# Autodesk Inventor assembly: Selection_Exit Pipe Assy 3 Lanes
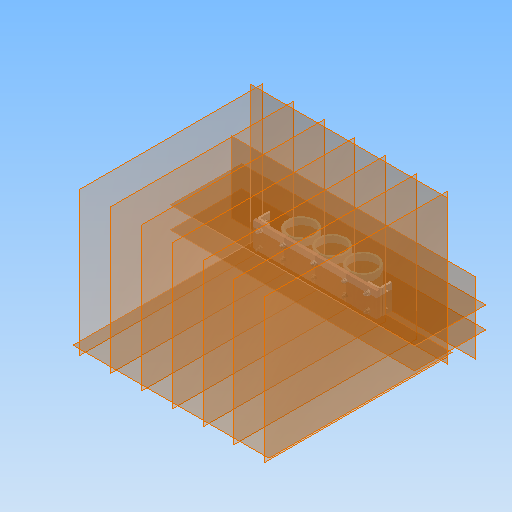
[picture p0: Inventor's stored thumbnail of the model, 512x512]
Saved by Autodesk Inventor 2018.1 (Build 221171000, 171)
## iProperties
Created: 2019-02-11
Part Number: Selection_Exit Pipe Assy 3 Lanes
Document SubType Name: Assembly
Designer: James
Author: James
## Documents named in this file (7)
- C:\Users\admin\Desktop\Ball-Machine\Selection Sort\Selection - 3 Lanes\Selection_Exit Pipe Assy 3 Lanes.iam
- C:\Users\admin\Desktop\Ball-Machine\Prototype CAD\Selection Sort - 40mm\Nyloc Nut - M4.ipt
- C:\Users\admin\Desktop\Ball-Machine\Prototype CAD\Selection Sort - 40mm\Socket Csk Screw - (A2) - M4 x  16.ipt
- C:\Users\admin\Desktop\Ball-Machine\Timing Gate\Timing_Angle Bracket.ipt
- C:\Users\admin\Desktop\Ball-Machine\Prototype CAD\Selection Sort - 40mm\Socket Cap Screw - Standard - (A2) - M4 x 16.ipt
- C:\Users\admin\Desktop\Ball-Machine\Selection Sort\Selection_Exit Pipe.ipt
- C:\Users\admin\Desktop\Ball-Machine\Timing Gate\Timing - 3 Lanes\Timing_Backboard 3 Lanes.ipt
## Components (26 placed, 6 different names)
1. Timing_Backboard 3 Lanes:1 — Flush:18, Tangent:1, Flush:19, Flush:20, Mate:55, Mate:56, Mate:59, Mate:60, Mate:67, Mate:68, Mate:69, Flush:27, Flush:28, Mate:74, Mate:75, Flush:29, Mate:82, Flush:30, Mate:83, Mate:84, Mate:85, Mate:88, Mate:89
2. Timing_Angle Bracket:1 — Mate:67, Mate:68, Mate:69, Flush:27, Flush:28, Mate:70, Mate:71, Mate:72, Mate:73
3. Nyloc Nut - M4:13 — Mate:74, Mate:76
4. Socket Cap Screw - Standard - (A2) - M4 x 16:3 — Mate:72, Mate:73, Mate:77
5. Nyloc Nut - M4:14 — Mate:75, Mate:77
6. Socket Cap Screw - Standard - (A2) - M4 x 16:4 — Mate:70, Mate:71, Mate:76
7. Timing_Angle Bracket:2 — Flush:29, Mate:82, Flush:30, Mate:83
8. Socket Cap Screw - Standard - (A2) - M4 x 16:5 — Mate:87
9. Socket Cap Screw - Standard - (A2) - M4 x 16:6 — Mate:86
10. Nyloc Nut - M4:15 — Mate:84, Mate:87
11. Nyloc Nut - M4:16 — Mate:85, Mate:86
12. Selection_Exit Pipe:1 — Tangent:1, Angle:1, Mate:88, Mate:89, Mate:90
13. Socket Csk Screw - (A2) - M4 x  16:1 — Mate:55, Flush:21, Mate:57, Mate:90
14. Nyloc Nut - M4:2 — Mate:57, Mate:60
15. Nyloc Nut - M4:1 — Mate:58, Mate:59
16. Socket Csk Screw - (A2) - M4 x  16:2 — Flush:21, Mate:56, Mate:58
17. Selection_Exit Pipe:2
18. Socket Csk Screw - (A2) - M4 x  16:3
19. Nyloc Nut - M4:17
20. Nyloc Nut - M4:18
21. Socket Csk Screw - (A2) - M4 x  16:4
22. Selection_Exit Pipe:3
23. Socket Csk Screw - (A2) - M4 x  16:5
24. Nyloc Nut - M4:19
25. Nyloc Nut - M4:20
26. Socket Csk Screw - (A2) - M4 x  16:6
## Component patterns: (3 elements, first: Selection_Exit Pipe:1 + Socket Csk Screw - (A2) - M4 x  16:1 + Nyloc Nut - M4:2 + Nyloc Nut - M4:1 + Socket Csk Screw - (A2) - M4 x  16:2)
## Relationships (43: Mate 30, Flush 11, Tangent 1, Angle 1)
- Flush:11 (-57.5 mm)
- Flush:12 (-5 mm)
- Flush:13 (30 mm)
- Flush:18: Timing_Backboard 3 Lanes:1
- Tangent:1: Timing_Backboard 3 Lanes:1 ↔ Selection_Exit Pipe:1
- Flush:19: Timing_Backboard 3 Lanes:1
- Flush:20: Timing_Backboard 3 Lanes:1
- Mate:55 (-10.3 mm): Timing_Backboard 3 Lanes:1 ↔ Socket Csk Screw - (A2) - M4 x  16:1
- Flush:21: Socket Csk Screw - (A2) - M4 x  16:1 ↔ Socket Csk Screw - (A2) - M4 x  16:2
- Mate:56: Timing_Backboard 3 Lanes:1 ↔ Socket Csk Screw - (A2) - M4 x  16:2
- Mate:57: Socket Csk Screw - (A2) - M4 x  16:1 ↔ Nyloc Nut - M4:2
- Mate:58: Nyloc Nut - M4:1 ↔ Socket Csk Screw - (A2) - M4 x  16:2
- Mate:59: Timing_Backboard 3 Lanes:1 ↔ Nyloc Nut - M4:1
- Mate:60: Timing_Backboard 3 Lanes:1 ↔ Nyloc Nut - M4:2
- Mate:67: Timing_Backboard 3 Lanes:1 ↔ Timing_Angle Bracket:1
- Mate:68: Timing_Backboard 3 Lanes:1 ↔ Timing_Angle Bracket:1
- Mate:69: Timing_Backboard 3 Lanes:1 ↔ Timing_Angle Bracket:1
- Flush:27: Timing_Backboard 3 Lanes:1 ↔ Timing_Angle Bracket:1
- Flush:28: Timing_Backboard 3 Lanes:1 ↔ Timing_Angle Bracket:1
- Mate:70: Timing_Angle Bracket:1 ↔ Socket Cap Screw - Standard - (A2) - M4 x 16:4
- Mate:71: Timing_Angle Bracket:1 ↔ Socket Cap Screw - Standard - (A2) - M4 x 16:4
- Mate:72: Timing_Angle Bracket:1 ↔ Socket Cap Screw - Standard - (A2) - M4 x 16:3
- Mate:73: Timing_Angle Bracket:1 ↔ Socket Cap Screw - Standard - (A2) - M4 x 16:3
- Mate:74: Timing_Backboard 3 Lanes:1 ↔ Nyloc Nut - M4:13
- Mate:75: Timing_Backboard 3 Lanes:1 ↔ Nyloc Nut - M4:14
- Mate:76: Nyloc Nut - M4:13 ↔ Socket Cap Screw - Standard - (A2) - M4 x 16:4
- Mate:77: Socket Cap Screw - Standard - (A2) - M4 x 16:3 ↔ Nyloc Nut - M4:14
- [Mate]: Timing_Angle Bracket:2 ↔ Socket Cap Screw - Standard - (A2) - M4 x 16:6
- [Mate]: Timing_Angle Bracket:2 ↔ Socket Cap Screw - Standard - (A2) - M4 x 16:6
- [Mate]: Timing_Angle Bracket:2 ↔ Socket Cap Screw - Standard - (A2) - M4 x 16:5
- [Mate]: Timing_Angle Bracket:2 ↔ Socket Cap Screw - Standard - (A2) - M4 x 16:5
- Flush:29: Timing_Backboard 3 Lanes:1 ↔ Timing_Angle Bracket:2
- Mate:82: Timing_Backboard 3 Lanes:1 ↔ Timing_Angle Bracket:2
- Flush:30: Timing_Backboard 3 Lanes:1 ↔ Timing_Angle Bracket:2
- Mate:83: Timing_Backboard 3 Lanes:1 ↔ Timing_Angle Bracket:2
- Mate:84: Timing_Backboard 3 Lanes:1 ↔ Nyloc Nut - M4:15
- Mate:85: Timing_Backboard 3 Lanes:1 ↔ Nyloc Nut - M4:16
- Mate:86: Socket Cap Screw - Standard - (A2) - M4 x 16:6 ↔ Nyloc Nut - M4:16
- Mate:87: Socket Cap Screw - Standard - (A2) - M4 x 16:5 ↔ Nyloc Nut - M4:15
- Angle:1 (0 deg): Selection_Exit Pipe:1
- Mate:88: Timing_Backboard 3 Lanes:1 ↔ Selection_Exit Pipe:1
- Mate:89: Timing_Backboard 3 Lanes:1 ↔ Selection_Exit Pipe:1
- Mate:90: Selection_Exit Pipe:1 ↔ Socket Csk Screw - (A2) - M4 x  16:1
## Named parameters: d139_d131 = 0 mm, d140_d132 = 0 mm, d141_d133 = 0 mm, d142_d134 = 0 mm
